# Autodesk Inventor assembly: Battery Cover
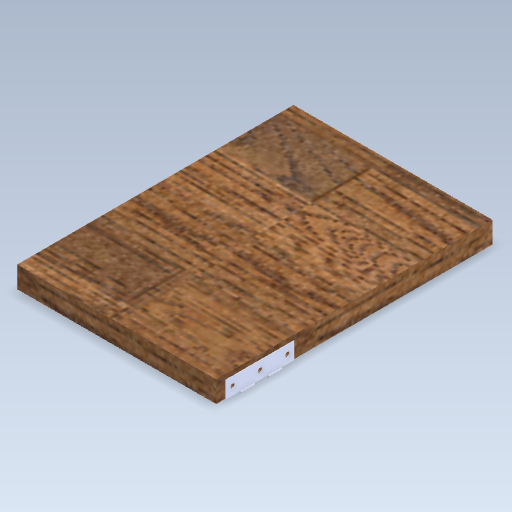
[picture p0: Inventor's stored thumbnail of the model, 512x512]
Saved by Autodesk Inventor 2020 (Build 240168000, 168)
## iProperties
Created: 2020-08-16
Part Number: Battery Cover
Document SubType Name: Assembly
Designer: Abbas
Author: Abbas
## Documents named in this file (3)
- C:\Users\LENOVO\Desktop\Graduation Project\Fish Farming Unit\Electric Box Covers\Battery Cover.iam
- C:\Users\LENOVO\Desktop\Graduation Project\Fish Farming Unit\Electric Box Covers\Battery Box Cover.ipt
- C:\Users\LENOVO\Desktop\Graduation Project\Fish Farming Unit\Hinge\Peice 2.ipt
## Components (2 placed, 2 different names)
1. Battery Box Cover:1 — Mate:1, Insert:1
2. Peice 2:1 — Mate:1, Insert:1
## Relationships (2: Mate 1, Insert 1)
- Mate:1: Battery Box Cover:1 ↔ Peice 2:1
- Insert:1: Battery Box Cover:1 ↔ Peice 2:1
